# Autodesk Inventor assembly: Temporizador
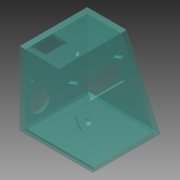
[picture p0: Inventor's stored thumbnail of the model, 180x180]
Saved by Autodesk Inventor 2014 (Build 180170000, 170)
## iProperties
Created: 2017-07-04
Part Number: Temporizador
Document SubType Name: Assembly
Designer: resaj
Author: resaj
## Documents named in this file (3)
- C:\Users\resaj\Dropbox\Proyectos\Temporizador\Temporizador.iam
- C:\Users\resaj\Dropbox\Proyectos\Temporizador\Caja temporizador.ipt
- C:\Users\resaj\Dropbox\Proyectos\Temporizador\Tapa.ipt
## Components (2 placed, 2 different names)
1. Caja temporizador:1 — Mate:1, Mate:2, Mate:3
2. Tapa:1 — Mate:1, Mate:2, Mate:3
## Relationships (3: Mate 3)
- Mate:1: Caja temporizador:1 ↔ Tapa:1
- Mate:2: Caja temporizador:1 ↔ Tapa:1
- Mate:3 (0.1 mm): Caja temporizador:1 ↔ Tapa:1
